# Autodesk Inventor assembly: Telaio - Taglio
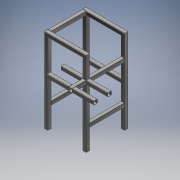
[picture p0: Inventor's stored thumbnail of the model, 180x180]
Saved by Autodesk Inventor 2018 (Build 220112000, 112)
## iProperties
Created: 2020-06-01
Part Number: Telaio - Taglio
Material: Generico
Document SubType Name: Assembly
Designer: Francesco
Author: Francesco
## Documents named in this file (7)
- C:\Users\Francesco\no-brim\Meccanica\Progetto Inventor no-brim\Assiemi\Telaio - Taglio.iam
- C:\Users\Francesco\no-brim\Meccanica\Progetto Inventor no-brim\Parti\Tubolare verticale 45 - Taglio.ipt
- C:\Users\Francesco\no-brim\Meccanica\Progetto Inventor no-brim\Parti\Tubolare horizontal 45 - Taglio.ipt
- C:\Users\Francesco\no-brim\Meccanica\Progetto Inventor no-brim\Parti\Tubolare horizontal - Taglio.ipt
- C:\Users\Francesco\no-brim\Meccanica\Progetto Inventor no-brim\Parti\Tubolare horizontal 2 - Taglio.ipt
- C:\Users\Francesco\no-brim\Meccanica\Progetto Inventor no-brim\Parti\Tubolari horizontal scarico.ipt
- C:\Users\Francesco\no-brim\Meccanica\Progetto Inventor no-brim\Parti\Tubolari horizontal scarico no 45.ipt
## Components (17 placed, 4 different names)
1. Tubolare verticale 45 - Taglio:1 — Coincidente:1, Allineato:1, Coincidente:2, Allineato:3, Coincidente:11, Allineato:10
2. Tubolare verticale 45 - Taglio:2 — Allineato:3, Coincidente:5, Allineato:4, Coincidente:6, Coincidente:12, Allineato:11, Coincidente:17, Allineato:18
3. Tubolare verticale 45 - Taglio:3 — Coincidente:7, Allineato:5, Coincidente:8, Allineato:8, Coincidente:14, Allineato:14, Coincidente:26, Allineato:36
4. Tubolare verticale 45 - Taglio:4 — Coincidente:3, Allineato:2, Coincidente:4, Coincidente:10, Coincidente:18, Allineato:21, Allineato:25, Coincidente:21, Coincidente:22, Allineato:27
5. Tubolare horizontal 45 - Taglio:1 — Coincidente:1, Allineato:1, Coincidente:2, Coincidente:3, Allineato:2, Coincidente:4, Allineato:6, Allineato:22, Allineato:35
6. Tubolare horizontal 45 - Taglio:2 — Coincidente:5, Allineato:4, Coincidente:6, Coincidente:7, Allineato:5, Coincidente:8, Allineato:6, Coincidente:9, Coincidente:25, Allineato:37
7. Tubolare horizontal - Taglio:1 — Coincidente:9, Allineato:8, Coincidente:10, Allineato:33
8. Tubolare horizontal - Taglio:2 — Coincidente:11, Allineato:10, Coincidente:15, Allineato:35
9. Tubolare horizontal - Taglio:3 — Coincidente:14, Allineato:14, Allineato:34
10. Tubolare horizontal - Taglio:5 — Coincidente:12, Allineato:11, Coincidente:15, Allineato:34
11. Tubolare horizontal - Taglio:7 — Coincidente:17, Allineato:18, Coincidente:25
12. Tubolari horizontal:1 — Coincidente:18, Allineato:21, Allineato:22, Allineato:24, Allineato:26, Coincidente:23, Allineato:29, Allineato:30, Coincidente:24, Allineato:31, Allineato:32
13. Tubolari horizontal:3 — Allineato:24, Allineato:25, Coincidente:21
14. Tubolari horizontal:4 — Coincidente:22, Allineato:26, Allineato:27, Allineato:33
15. Tubolari horizontal:5 — Coincidente:23, Allineato:29, Allineato:30
16. Tubolari horizontal:6 — Coincidente:24, Allineato:31, Allineato:32
17. Tubolare horizontal - Taglio:8 — Coincidente:26, Allineato:36, Allineato:37
## Relationships (48: Flush 26, Mate 22)
- Coincidente:1 [Mate]: Tubolare verticale 45 - Taglio:1 ↔ Tubolare horizontal 45 - Taglio:1
- Allineato:1 [Flush]: Tubolare verticale 45 - Taglio:1 ↔ Tubolare horizontal 45 - Taglio:1
- Coincidente:2 [Mate]: Tubolare verticale 45 - Taglio:1 ↔ Tubolare horizontal 45 - Taglio:1
- Coincidente:3 [Mate]: Tubolare verticale 45 - Taglio:4 ↔ Tubolare horizontal 45 - Taglio:1
- Allineato:2 [Flush]: Tubolare verticale 45 - Taglio:4 ↔ Tubolare horizontal 45 - Taglio:1
- Coincidente:4 [Mate]: Tubolare verticale 45 - Taglio:4 ↔ Tubolare horizontal 45 - Taglio:1
- Allineato:3 [Flush]: Tubolare verticale 45 - Taglio:1 ↔ Tubolare verticale 45 - Taglio:2
- Coincidente:5 [Mate]: Tubolare verticale 45 - Taglio:2 ↔ Tubolare horizontal 45 - Taglio:2
- Allineato:4 [Flush]: Tubolare verticale 45 - Taglio:2 ↔ Tubolare horizontal 45 - Taglio:2
- Coincidente:6 [Mate]: Tubolare verticale 45 - Taglio:2 ↔ Tubolare horizontal 45 - Taglio:2
- Coincidente:7 [Mate]: Tubolare verticale 45 - Taglio:3 ↔ Tubolare horizontal 45 - Taglio:2
- Allineato:5 [Flush]: Tubolare verticale 45 - Taglio:3 ↔ Tubolare horizontal 45 - Taglio:2
- Coincidente:8 [Mate]: Tubolare verticale 45 - Taglio:3 ↔ Tubolare horizontal 45 - Taglio:2
- Allineato:6 [Flush]: Tubolare horizontal 45 - Taglio:1 ↔ Tubolare horizontal 45 - Taglio:2
- Coincidente:9 [Mate]: Tubolare horizontal 45 - Taglio:2 ↔ Tubolare horizontal - Taglio:1
- Allineato:8 [Flush]: Tubolare verticale 45 - Taglio:3 ↔ Tubolare horizontal - Taglio:1
- Coincidente:10 [Mate]: Tubolare verticale 45 - Taglio:4 ↔ Tubolare horizontal - Taglio:1
- Coincidente:11 [Mate]: Tubolare verticale 45 - Taglio:1 ↔ Tubolare horizontal - Taglio:2
- Allineato:10 [Flush]: Tubolare verticale 45 - Taglio:1 ↔ Tubolare horizontal - Taglio:2
- Coincidente:12 [Mate]: Tubolare verticale 45 - Taglio:2 ↔ Tubolare horizontal - Taglio:5
- Allineato:11 [Flush]: Tubolare verticale 45 - Taglio:2 ↔ Tubolare horizontal - Taglio:5
- Coincidente:14 [Mate]: Tubolare verticale 45 - Taglio:3 ↔ Tubolare horizontal - Taglio:3
- Allineato:14 [Flush]: Tubolare verticale 45 - Taglio:3 ↔ Tubolare horizontal - Taglio:3
- Coincidente:15 [Mate] (607.5 mm): Tubolare horizontal - Taglio:2 ↔ Tubolare horizontal - Taglio:5
- Coincidente:17 [Mate]: Tubolare verticale 45 - Taglio:2 ↔ Tubolare horizontal - Taglio:7
- Allineato:18 [Flush]: Tubolare verticale 45 - Taglio:2 ↔ Tubolare horizontal - Taglio:7
- Coincidente:18 [Mate]: Tubolare verticale 45 - Taglio:4 ↔ Tubolari horizontal:1
- Allineato:21 [Flush]: Tubolare verticale 45 - Taglio:4 ↔ Tubolari horizontal:1
- Allineato:22 [Flush] (232 mm): Tubolare horizontal 45 - Taglio:1 ↔ Tubolari horizontal:1
- Allineato:24 [Flush]: Tubolari horizontal:1 ↔ Tubolari horizontal:3
- Allineato:25 [Flush]: Tubolare verticale 45 - Taglio:4 ↔ Tubolari horizontal:3
- Coincidente:21 [Mate]: Tubolare verticale 45 - Taglio:4 ↔ Tubolari horizontal:3
- Coincidente:22 [Mate]: Tubolare verticale 45 - Taglio:4 ↔ Tubolari horizontal:4
- Allineato:26 [Flush]: Tubolari horizontal:1 ↔ Tubolari horizontal:4
- Allineato:27 [Flush]: Tubolare verticale 45 - Taglio:4 ↔ Tubolari horizontal:4
- Coincidente:23 [Mate]: Tubolari horizontal:1 ↔ Tubolari horizontal:5
- Allineato:29 [Flush]: Tubolari horizontal:1 ↔ Tubolari horizontal:5
- Allineato:30 [Flush]: Tubolari horizontal:1 ↔ Tubolari horizontal:5
- Coincidente:24 [Mate]: Tubolari horizontal:1 ↔ Tubolari horizontal:6
- Allineato:31 [Flush]: Tubolari horizontal:1 ↔ Tubolari horizontal:6
- Allineato:32 [Flush]: Tubolari horizontal:1 ↔ Tubolari horizontal:6
- Allineato:33 [Flush]: Tubolare horizontal - Taglio:1 ↔ Tubolari horizontal:4
- Coincidente:25 [Mate] (400 mm): Tubolare horizontal 45 - Taglio:2 ↔ Tubolare horizontal - Taglio:7
- Allineato:34 [Flush]: Tubolare horizontal - Taglio:3 ↔ Tubolare horizontal - Taglio:5
- Allineato:35 [Flush]: Tubolare horizontal 45 - Taglio:1 ↔ Tubolare horizontal - Taglio:2
- Coincidente:26 [Mate]: Tubolare verticale 45 - Taglio:3 ↔ Tubolare horizontal - Taglio:8
- Allineato:36 [Flush]: Tubolare verticale 45 - Taglio:3 ↔ Tubolare horizontal - Taglio:8
- Allineato:37 [Flush]: Tubolare horizontal 45 - Taglio:2 ↔ Tubolare horizontal - Taglio:8
